# Autodesk Inventor assembly: ext_GLS Assembly
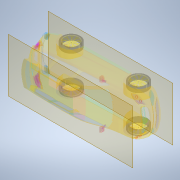
[picture p0: Inventor's stored thumbnail of the model, 180x180]
Saved by Autodesk Inventor 2021 (Build 250183000, 183)
## iProperties
Company: DESKTOP-R9FR9R7
Created: 2021-03-19
Part Number: ext_GLS Assembly
Description: START RECORD GO HERE.
Document SubType Name: Assembly
Designer: Watchdog
Sending System: DASSAULT SYSTEMES CATIA V5 R20 - www.3ds.com
Preprocessor: CATIA Version 5 Release 20
Minimum Resolution: 0.001
Sending System Product ID: Product1
Receiving System Product ID: Product1
Sent Units: Millimeter
Translation Standard: IGES 5.3
Model Creation Time: 2021-03-19
Title: GLS Assembly.igs
Author: c
## Documents named in this file (4)
- C:\Users\ocon0143\OneDrive - Flinders\Advn Mech Design Shared\6_Development\2_Design\inventor\vehicle_wheelchair\mb_gls\ext_GLS Assembly.iam
- C:\Users\ocon0143\OneDrive - Flinders\Advn Mech Design Shared\6_Development\2_Design\inventor\vehicle_wheelchair\mb_gls\ext_Assembly2.iam
- C:\Users\ocon0143\OneDrive - Flinders\Advn Mech Design Shared\6_Development\2_Design\inventor\vehicle_wheelchair\mb_gls\ext_Part4.ipt
- C:\Users\ocon0143\OneDrive - Flinders\Advn Mech Design Shared\6_Development\2_Design\inventor\vehicle_wheelchair\mb_gls\ext_Part1.1.ipt
## Components (7 placed, 7 different names)
1. Product1.1 [sub-assembly] — Mate:1, Mate:2
2. Part4.1
3. Part4.2
4. Part1.1
5. Part1.2
6. Part1.3 — Tangent:1
7. Part1.4
## Relationships (7: Angle 3, Mate 2, Tangent 1, Flush 1)
- Angle:1 (0 deg)
- Tangent:1: Part1.3
- Mate:1: Product1.1
- Angle:2 (0 deg)
- Mate:2: Product1.1
- Angle:3 (0 deg)
- Flush:1 (1800 mm)
